# Autodesk Inventor assembly: Cylinder
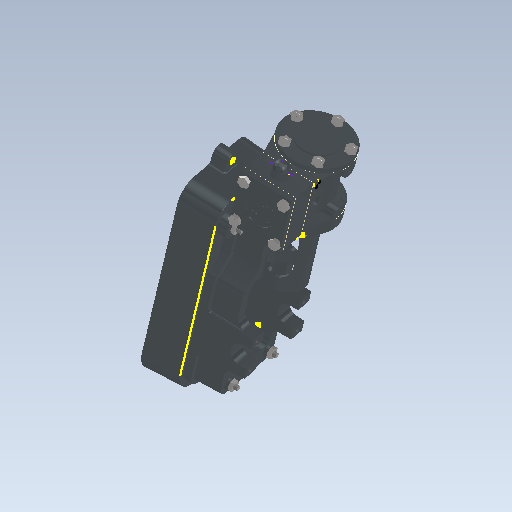
[picture p0: Inventor's stored thumbnail of the model, 512x512]
Saved by Autodesk Inventor 2020 (Build 240168000, 168)
## iProperties
Created: 2021-10-26
Part Number: Cylinder
Document SubType Name: Assembly
Designer: simon.erikssonwestl
Author: simon.erikssonwestl
## Documents named in this file (14)
- C:\Users\simon.erikssonwestl\Documents\Inventor\Ång\Assemblies\Cylinder.iam
- C:\Users\simon.erikssonwestl\Documents\Inventor\Ång\Part1.ipt
- C:\Users\simon.erikssonwestl\Documents\Inventor\Ång\Part2.ipt
- C:\Users\simon.erikssonwestl\Documents\Inventor\Content Center Files\R2020\en-US\DIN 976-1 A\DIN 976-1 - M2,5 x 25 - A.ipt
- C:\Users\simon.erikssonwestl\Documents\Inventor\Content Center Files\R2020\en-US\DIN 976-1 A\DIN 976-1 - M2,5 x 12 - A.ipt
- C:\Users\simon.erikssonwestl\Documents\Inventor\Content Center Files\R2020\en-US\AS 1474(1)\AS 1474 - M2,5(1).ipt
- C:\Users\simon.erikssonwestl\Documents\Inventor\Ång\Part9.ipt
- C:\Users\simon.erikssonwestl\Documents\Inventor\Content Center Files\R2020\en-US\DIN 976-1 A\DIN 976-1 - M2,5 x 10 - A.ipt
- C:\Users\simon.erikssonwestl\Documents\Inventor\Ång\Part7.ipt
- C:\Users\simon.erikssonwestl\Documents\Inventor\Ång\Part3.ipt
- C:\Users\simon.erikssonwestl\Documents\Inventor\Ång\Part10.ipt
- C:\Users\simon.erikssonwestl\Documents\Inventor\Ång\Part6.ipt
- C:\Users\simon.erikssonwestl\Documents\Inventor\Ång\Part4.ipt
- C:\Users\simon.erikssonwestl\Documents\Inventor\Ång\Part5.ipt
## Components (47 placed, 13 different names)
1. Part1:1 — Mate:3, Mate:4, Mate:7, Mate:8, Flush:1, Flush:2, Flush:3, Flush:4, Mate:11
2. Part2:1 — Mate:5, Mate:6, Mate:9, Mate:10, Mate:11, Mate:16, Mate:17, Mate:18, Mate:19, Mate:20, Mate:21, Mate:22, Mate:23, Mate:24, Mate:25, Mate:31, Mate:45, Mate:50, Mate:51, Mate:52, Mate:53
3. DIN 976-1 A M2,5 x 25:1 — Mate:8, Mate:10, Flush:4, Mate:14
4. DIN 976-1 A M2,5 x 25:2 — Mate:7, Mate:9, Flush:3, Mate:15
5. DIN 976-1 A M2,5 x 12:1 — Mate:4, Mate:5, Flush:1, Mate:13
6. DIN 976-1 A M2,5 x 12:2 — Mate:3, Mate:6, Flush:2, Mate:12
7. AS 1474 - Metric M2,5:1 — Mate:12, Mate:16
8. AS 1474 - Metric M2,5:2 — Mate:13, Mate:17
9. AS 1474 - Metric M2,5:3 — Mate:14, Mate:18
10. AS 1474 - Metric M2,5:4 — Mate:15, Mate:19
11. Part9:1 — Mate:20, Mate:26, Mate:27, Mate:28, Mate:29, Mate:30, Mate:31, Mate:38
12. DIN 976-1 A M2,5 x 10:1 — Mate:21, Mate:27, Mate:33, Mate:48, Flush:7
13. DIN 976-1 A M2,5 x 10:2 — Mate:22, Mate:26, Mate:32, Mate:37, Mate:40, Mate:49, Flush:6
14. DIN 976-1 A M2,5 x 10:3 — Mate:23, Mate:30, Mate:36, Mate:41, Mate:44, Flush:5
15. DIN 976-1 A M2,5 x 10:4 — Mate:24, Mate:29, Mate:35, Mate:42, Mate:46, Flush:9
16. DIN 976-1 A M2,5 x 10:5 — Mate:25, Mate:28, Mate:34, Mate:43, Mate:47, Flush:8
17. Part7:1 — Mate:32, Mate:33, Mate:34, Mate:35, Mate:36, Mate:37, Mate:38, Mate:54
18. Part3:1 — Mate:40, Mate:41, Mate:42, Mate:43, Mate:54, Mate:55, Mate:56, Mate:57, Mate:58, Mate:59, Mate:62, Mate:76, Mate:77, Mate:78, Mate:79, Mate:82
19. AS 1474 - Metric M2,5:5 — Mate:44, Mate:45, Flush:5
20. AS 1474 - Metric M2,5:6 — Mate:46, Mate:53, Flush:9
21. AS 1474 - Metric M2,5:7 — Mate:47, Mate:52, Flush:8
22. AS 1474 - Metric M2,5:8 — Mate:48, Mate:51, Flush:7
23. AS 1474 - Metric M2,5:9 — Mate:49, Mate:50, Flush:6
24. Part7:2 — Mate:60, Mate:61, Mate:62, Mate:75
25. Part10:1 — Mate:63, Mate:64, Mate:70, Mate:71, Mate:72, Mate:73, Mate:74, Mate:75
26. DIN 976-1 A M2,5 x 10:6 — Mate:59, Mate:69, Flush:12
27. DIN 976-1 A M2,5 x 10:7 — Mate:58, Mate:64, Mate:66, Flush:11
28. DIN 976-1 A M2,5 x 10:8 — Mate:57, Mate:60, Mate:63, Mate:65, Flush:10
29. DIN 976-1 A M2,5 x 10:9 — Mate:56, Mate:61, Mate:67, Flush:14
30. DIN 976-1 A M2,5 x 10:10 — Mate:55, Mate:68, Flush:13
31. AS 1474 - Metric M2,5:10 — Mate:69, Mate:74, Flush:12
32. AS 1474 - Metric M2,5:11 — Mate:68, Mate:73, Flush:13
33. AS 1474 - Metric M2,5:12 — Mate:67, Mate:72, Flush:14
34. AS 1474 - Metric M2,5:13 — Mate:66, Mate:70, Flush:11
35. AS 1474 - Metric M2,5:14 — Mate:65, Mate:71, Flush:10
36. DIN 976-1 A M2,5 x 25:3 — Mate:76, Mate:83, Mate:89, Mate:92, Flush:18
37. DIN 976-1 A M2,5 x 25:4 — Mate:77, Mate:81, Mate:87, Mate:93, Flush:17
38. DIN 976-1 A M2,5 x 25:5 — Mate:78, Mate:80, Mate:86, Mate:94, Flush:15
39. DIN 976-1 A M2,5 x 25:6 — Mate:79, Mate:84, Mate:90, Mate:95, Flush:16
40. Part6:1 — Mate:86, Mate:87, Mate:88, Mate:91
41. Part6:2 — Mate:80, Mate:81, Mate:82, Mate:85
42. Part4:1 — Mate:83, Mate:84, Mate:85, Mate:88
43. Part5:1 — Mate:89, Mate:90, Mate:91, Mate:96, Mate:97, Mate:98, Mate:99
44. AS 1474 - Metric M2,5:15 — Mate:95, Mate:96, Flush:16
45. AS 1474 - Metric M2,5:16 — Mate:94, Mate:97, Flush:15
46. AS 1474 - Metric M2,5:17 — Mate:93, Mate:99, Flush:17
47. AS 1474 - Metric M2,5:18 — Mate:92, Mate:98, Flush:18
## Relationships (114: Mate 96, Flush 18)
- Mate:3: Part1:1 ↔ DIN 976-1 A M2,5 x 12:2
- Mate:4: Part1:1 ↔ DIN 976-1 A M2,5 x 12:1
- Mate:5: Part2:1 ↔ DIN 976-1 A M2,5 x 12:1
- Mate:6: Part2:1 ↔ DIN 976-1 A M2,5 x 12:2
- Mate:7: Part1:1 ↔ DIN 976-1 A M2,5 x 25:2
- Mate:8: Part1:1 ↔ DIN 976-1 A M2,5 x 25:1
- Mate:9: Part2:1 ↔ DIN 976-1 A M2,5 x 25:2
- Mate:10: Part2:1 ↔ DIN 976-1 A M2,5 x 25:1
- Flush:1: Part1:1 ↔ DIN 976-1 A M2,5 x 12:1
- Flush:2: Part1:1 ↔ DIN 976-1 A M2,5 x 12:2
- Flush:3: Part1:1 ↔ DIN 976-1 A M2,5 x 25:2
- Flush:4: Part1:1 ↔ DIN 976-1 A M2,5 x 25:1
- Mate:11: Part1:1 ↔ Part2:1
- Mate:12: DIN 976-1 A M2,5 x 12:2 ↔ AS 1474 - Metric M2,5:1
- Mate:13: DIN 976-1 A M2,5 x 12:1 ↔ AS 1474 - Metric M2,5:2
- Mate:14: DIN 976-1 A M2,5 x 25:1 ↔ AS 1474 - Metric M2,5:3
- Mate:15: DIN 976-1 A M2,5 x 25:2 ↔ AS 1474 - Metric M2,5:4
- Mate:16: Part2:1 ↔ AS 1474 - Metric M2,5:1
- Mate:17: Part2:1 ↔ AS 1474 - Metric M2,5:2
- Mate:18: Part2:1 ↔ AS 1474 - Metric M2,5:3
- Mate:19: Part2:1 ↔ AS 1474 - Metric M2,5:4
- Mate:20: Part2:1 ↔ Part9:1
- Mate:21: Part2:1 ↔ DIN 976-1 A M2,5 x 10:1
- Mate:22: Part2:1 ↔ DIN 976-1 A M2,5 x 10:2
- Mate:23: Part2:1 ↔ DIN 976-1 A M2,5 x 10:3
- Mate:24: Part2:1 ↔ DIN 976-1 A M2,5 x 10:4
- Mate:25: Part2:1 ↔ DIN 976-1 A M2,5 x 10:5
- Mate:26: Part9:1 ↔ DIN 976-1 A M2,5 x 10:2
- Mate:27: Part9:1 ↔ DIN 976-1 A M2,5 x 10:1
- Mate:28: Part9:1 ↔ DIN 976-1 A M2,5 x 10:5
- Mate:29: Part9:1 ↔ DIN 976-1 A M2,5 x 10:4
- Mate:30: Part9:1 ↔ DIN 976-1 A M2,5 x 10:3
- Mate:31: Part2:1 ↔ Part9:1
- Mate:32: DIN 976-1 A M2,5 x 10:2 ↔ Part7:1
- Mate:33: DIN 976-1 A M2,5 x 10:1 ↔ Part7:1
- Mate:34: DIN 976-1 A M2,5 x 10:5 ↔ Part7:1
- Mate:35: DIN 976-1 A M2,5 x 10:4 ↔ Part7:1
- Mate:36: DIN 976-1 A M2,5 x 10:3 ↔ Part7:1
- Mate:37: DIN 976-1 A M2,5 x 10:2 ↔ Part7:1
- Mate:38: Part9:1 ↔ Part7:1
- Mate:40: DIN 976-1 A M2,5 x 10:2 ↔ Part3:1
- Mate:41: DIN 976-1 A M2,5 x 10:3 ↔ Part3:1
- Mate:42: DIN 976-1 A M2,5 x 10:4 ↔ Part3:1
- Mate:43: DIN 976-1 A M2,5 x 10:5 ↔ Part3:1
- Mate:44: DIN 976-1 A M2,5 x 10:3 ↔ AS 1474 - Metric M2,5:5
- Mate:45: Part2:1 ↔ AS 1474 - Metric M2,5:5
- Flush:5: DIN 976-1 A M2,5 x 10:3 ↔ AS 1474 - Metric M2,5:5
- Mate:46: DIN 976-1 A M2,5 x 10:4 ↔ AS 1474 - Metric M2,5:6
- Mate:47: DIN 976-1 A M2,5 x 10:5 ↔ AS 1474 - Metric M2,5:7
- Mate:48: DIN 976-1 A M2,5 x 10:1 ↔ AS 1474 - Metric M2,5:8
- Mate:49: DIN 976-1 A M2,5 x 10:2 ↔ AS 1474 - Metric M2,5:9
- Mate:50: Part2:1 ↔ AS 1474 - Metric M2,5:9
- Mate:51: Part2:1 ↔ AS 1474 - Metric M2,5:8
- Mate:52: Part2:1 ↔ AS 1474 - Metric M2,5:7
- Mate:53: Part2:1 ↔ AS 1474 - Metric M2,5:6
- Flush:6: DIN 976-1 A M2,5 x 10:2 ↔ AS 1474 - Metric M2,5:9
- Flush:7: DIN 976-1 A M2,5 x 10:1 ↔ AS 1474 - Metric M2,5:8
- Flush:8: DIN 976-1 A M2,5 x 10:5 ↔ AS 1474 - Metric M2,5:7
- Flush:9: DIN 976-1 A M2,5 x 10:4 ↔ AS 1474 - Metric M2,5:6
- Mate:54: Part7:1 ↔ Part3:1
- Mate:55: Part3:1 ↔ DIN 976-1 A M2,5 x 10:10
- Mate:56: Part3:1 ↔ DIN 976-1 A M2,5 x 10:9
- Mate:57: Part3:1 ↔ DIN 976-1 A M2,5 x 10:8
- Mate:58: Part3:1 ↔ DIN 976-1 A M2,5 x 10:7
- Mate:59: Part3:1 ↔ DIN 976-1 A M2,5 x 10:6
- Mate:60: Part7:2 ↔ DIN 976-1 A M2,5 x 10:8
- Mate:61: Part7:2 ↔ DIN 976-1 A M2,5 x 10:9
- Mate:62: Part3:1 ↔ Part7:2
- Mate:63: Part10:1 ↔ DIN 976-1 A M2,5 x 10:8
- Mate:64: Part10:1 ↔ DIN 976-1 A M2,5 x 10:7
- Mate:65: DIN 976-1 A M2,5 x 10:8 ↔ AS 1474 - Metric M2,5:14
- Mate:66: DIN 976-1 A M2,5 x 10:7 ↔ AS 1474 - Metric M2,5:13
- Mate:67: DIN 976-1 A M2,5 x 10:9 ↔ AS 1474 - Metric M2,5:12
- Mate:68: DIN 976-1 A M2,5 x 10:10 ↔ AS 1474 - Metric M2,5:11
- Mate:69: DIN 976-1 A M2,5 x 10:6 ↔ AS 1474 - Metric M2,5:10
- Mate:70: Part10:1 ↔ AS 1474 - Metric M2,5:13
- Mate:71: Part10:1 ↔ AS 1474 - Metric M2,5:14
- Mate:72: Part10:1 ↔ AS 1474 - Metric M2,5:12
- Mate:73: Part10:1 ↔ AS 1474 - Metric M2,5:11
- Mate:74: Part10:1 ↔ AS 1474 - Metric M2,5:10
- Flush:10: DIN 976-1 A M2,5 x 10:8 ↔ AS 1474 - Metric M2,5:14
- Flush:11: DIN 976-1 A M2,5 x 10:7 ↔ AS 1474 - Metric M2,5:13
- Flush:12: DIN 976-1 A M2,5 x 10:6 ↔ AS 1474 - Metric M2,5:10
- Flush:13: DIN 976-1 A M2,5 x 10:10 ↔ AS 1474 - Metric M2,5:11
- Flush:14: DIN 976-1 A M2,5 x 10:9 ↔ AS 1474 - Metric M2,5:12
- Mate:75: Part7:2 ↔ Part10:1
- Mate:76: Part3:1 ↔ DIN 976-1 A M2,5 x 25:3
- Mate:77: Part3:1 ↔ DIN 976-1 A M2,5 x 25:4
- Mate:78: Part3:1 ↔ DIN 976-1 A M2,5 x 25:5
- Mate:79: Part3:1 ↔ DIN 976-1 A M2,5 x 25:6
- Mate:80: DIN 976-1 A M2,5 x 25:5 ↔ Part6:2
- Mate:81: DIN 976-1 A M2,5 x 25:4 ↔ Part6:2
- Mate:82: Part3:1 ↔ Part6:2
- Mate:83: DIN 976-1 A M2,5 x 25:3 ↔ Part4:1
- Mate:84: DIN 976-1 A M2,5 x 25:6 ↔ Part4:1
- Mate:85: Part6:2 ↔ Part4:1
- Mate:86: DIN 976-1 A M2,5 x 25:5 ↔ Part6:1
- Mate:87: DIN 976-1 A M2,5 x 25:4 ↔ Part6:1
- Mate:88: Part6:1 ↔ Part4:1
- Mate:89: DIN 976-1 A M2,5 x 25:3 ↔ Part5:1
- Mate:90: DIN 976-1 A M2,5 x 25:6 ↔ Part5:1
- Mate:91: Part6:1 ↔ Part5:1
- Mate:92: DIN 976-1 A M2,5 x 25:3 ↔ AS 1474 - Metric M2,5:18
- Mate:93: DIN 976-1 A M2,5 x 25:4 ↔ AS 1474 - Metric M2,5:17
- Mate:94: DIN 976-1 A M2,5 x 25:5 ↔ AS 1474 - Metric M2,5:16
- Mate:95: DIN 976-1 A M2,5 x 25:6 ↔ AS 1474 - Metric M2,5:15
- Mate:96: Part5:1 ↔ AS 1474 - Metric M2,5:15
- Mate:97: Part5:1 ↔ AS 1474 - Metric M2,5:16
- Mate:98: Part5:1 ↔ AS 1474 - Metric M2,5:18
- Mate:99: Part5:1 ↔ AS 1474 - Metric M2,5:17
- Flush:15: DIN 976-1 A M2,5 x 25:5 ↔ AS 1474 - Metric M2,5:16
- Flush:16: DIN 976-1 A M2,5 x 25:6 ↔ AS 1474 - Metric M2,5:15
- Flush:17: DIN 976-1 A M2,5 x 25:4 ↔ AS 1474 - Metric M2,5:17
- Flush:18: DIN 976-1 A M2,5 x 25:3 ↔ AS 1474 - Metric M2,5:18
